# Autodesk Inventor assembly: Ensamblaje1
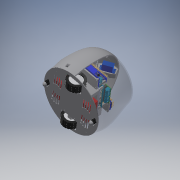
[picture p0: Inventor's stored thumbnail of the model, 180x180]
Saved by Autodesk Inventor 2018 (Build 220112000, 112)
## iProperties
Created: 2018-02-22
Part Number: Ensamblaje1
Material: Genérico
Document SubType Name: Assembly
Designer: ivanb
Author: ivanb
## Documents named in this file (22)
- C:\Users\ivanb\learnbot-git-annex\learnbot_desings\Learnbot2.1\IPT\Learnbot2.0.iam
- C:\Users\ivanb\learnbot-git-annex\learnbot_desings\Learnbot2.1\IPT\Base.ipt
- C:\Users\ivanb\learnbot-git-annex\learnbot_desings\Learnbot2.1\IPT\BackCase.ipt
- C:\Users\ivanb\learnbot-git-annex\learnbot_desings\Learnbot2.1\IPT\Front Case.ipt
- C:\Users\ivanb\learnbot-git-annex\learnbot_desings\Learnbot2.0\filesToPrintLearnbot\IPT\carcasa_camara2.0.ipt
- C:\Users\ivanb\learnbot-git-annex\servo motor.ipt
- C:\Users\ivanb\learnbot-git-annex\learnbot_desings\Learnbot2.1\IPT\Wheel.ipt
- C:\Users\ivanb\learnbot-git-annex\learnbot_desings\Learnbot2.1\IPT\Caster ball.ipt
- C:\Users\ivanb\learnbot-git-annex\learnbot_desings\Learnbot2.1\IPT\Servo Pulley.ipt
- C:\Users\ivanb\learnbot-git-annex\learnbot_desings\Learnbot2.1\IPT\Cover camera case.ipt
- C:\Users\ivanb\learnbot-git-annex\learnbot_desings\Learnbot2.1\IPT\raspberrypi.ipt
- C:\Users\ivanb\learnbot-git-annex\learnbot_desings\Learnbot2.1\IPT\Soport Raspberry.ipt
- C:\Users\ivanb\learnbot-git-annex\learnbot_desings\Learnbot2.1\IPT\Pitft 3.5.ipt
- C:\Users\ivanb\learnbot-git-annex\learnbot_desings\Learnbot2.1\IPT\Expansion-Extension.ipt
- C:\Users\ivanb\learnbot-git-annex\learnbot_desings\Learnbot2.1\IPT\Spacer 3mm.ipt
- C:\Users\ivanb\learnbot-git-annex\learnbot_desings\Learnbot2.1\IPT\pololu 8835.ipt
- C:\Users\ivanb\learnbot-git-annex\learnbot_desings\Learnbot2.1\IPT\Voltage regulator.ipt
- C:\Users\ivanb\learnbot-git-annex\learnbot_desings\Learnbot2.1\IPT\Spacer 19.5 mm.ipt
- C:\Users\ivanb\learnbot-git-annex\learnbot_desings\Learnbot2.1\IPT\Pin multiplier.ipt
- C:\Users\ivanb\learnbot-git-annex\learnbot_desings\Learnbot2.1\IPT\Batery.ipt
- C:\Users\ivanb\learnbot-git-annex\learnbot_desings\Learnbot2.1\IPT\Board 16 pwm.ipt
- C:\Users\ivanb\learnbot-git-annex\learnbot_desings\Learnbot2.1\IPT\Soport 16 pwm.ipt
## Components (27 placed, 21 different names)
1. Base:1 — Coincidencia:1, Insertar:1, Insertar:2, Coincidencia:2, Coincidencia:5, Coincidencia:6, Insertar:11, Insertar:12, Insertar:13, Insertar:14, Insertar:29, Insertar:30, Insertar:32, Insertar:33, Insertar:34, Insertar:35, Coincidencia:12
2. Front Case:1 — Coincidencia:1, Insertar:1, Insertar:2, Insertar:6, Insertar:7, Insertar:8, Insertar:10, Insertar:19, Insertar:28, Insertar:29, Insertar:30, Coincidencia:14, Coincidencia:15, Coincidencia:16
3. BackCase:1 — Coincidencia:2, Insertar:32, Insertar:33
4. carcasa_camara2.0:1 — Nivelación:2, Insertar:8, Coincidencia:7, Insertar:9, Insertar:10, Insertar:19, Rígido:3, Insertar:20
5. servo motor:1 — Nivelación:2, Insertar:6, Insertar:7, De rotación:1, Insertar:28
6. Wheel:1 — Rígido:5
7. Wheel:2 — Rígido:4
8. Caster ball:1 — Coincidencia:6, Insertar:11, Insertar:12
9. Caster ball:2 — Coincidencia:5, Insertar:13, Insertar:14
10. Servo Pulley:1 — De rotación:1
11. Cover camera case:1 — Coincidencia:7, Insertar:9, Rígido:3, Insertar:20
12. Pitft 3.5:1 — Coincidencia:14, Coincidencia:15, Coincidencia:16
13. Soport Raspberry:1 — Insertar:34, Insertar:35, Rígido:4, Rígido:5, Insertar:36, Insertar:37, Insertar:50, Insertar:51, Coincidencia:13
14. raspberrypi:1 — Insertar:36, Insertar:37, Tangente:1, Tangente:2, Coincidencia:10, Insertar:38, Insertar:39, Insertar:40, Insertar:41
15. Expansion-Extension:1 — Tangente:1, Tangente:2, Coincidencia:10, Coincidencia:11, Rígido:6, Insertar:52, Insertar:53
16. Spacer 3mm:1 — Insertar:38
17. Spacer 3mm:2 — Insertar:39
18. Spacer 3mm:3 — Insertar:41
19. Spacer 3mm:4 — Insertar:40
20. pololu 8835:1 — Coincidencia:11, Rígido:6
21. Voltage regulator:1 — Insertar:46, Insertar:47, Insertar:50, Insertar:51
22. Spacer 19.5 mm:3 — Insertar:46, Insertar:48
23. Spacer 19.5 mm:4 — Insertar:47, Insertar:49
24. Pin multiplier:1 — Insertar:48, Insertar:49
25. Batery:1 — Coincidencia:12, Coincidencia:13
26. Board 16 pwm:1 — Insertar:54, Insertar:55
27. Soport 16 pwm:1 — Insertar:52, Insertar:53, Insertar:54, Insertar:55
## Relationships (56: Insert 36, Mate 12, WeldJoint 4, Tangent 2, Flush 1, RevoluteJoint 1)
- Coincidencia:1 [Mate]: Base:1 ↔ Front Case:1
- Insertar:1: Base:1 ↔ Front Case:1
- Insertar:2: Base:1 ↔ Front Case:1
- Coincidencia:2 [Mate]: Base:1 ↔ BackCase:1
- Nivelación:2 [Flush]: carcasa_camara2.0:1 ↔ servo motor:1
- Insertar:6: Front Case:1 ↔ servo motor:1
- Insertar:7: Front Case:1 ↔ servo motor:1
- Coincidencia:5 [Mate]: Base:1 ↔ Caster ball:2
- Coincidencia:6 [Mate]: Base:1 ↔ Caster ball:1
- Insertar:8: Front Case:1 ↔ carcasa_camara2.0:1
- De rotación:1 [RevoluteJoint]: servo motor:1 ↔ Servo Pulley:1
- Coincidencia:7 [Mate]: carcasa_camara2.0:1 ↔ Cover camera case:1
- Insertar:9: carcasa_camara2.0:1 ↔ Cover camera case:1
- Insertar:10: Front Case:1 ↔ carcasa_camara2.0:1
- Insertar:11: Base:1 ↔ Caster ball:1
- Insertar:12: Base:1 ↔ Caster ball:1
- Insertar:13: Base:1 ↔ Caster ball:2
- Insertar:14: Base:1 ↔ Caster ball:2
- Insertar:19: Front Case:1 ↔ carcasa_camara2.0:1
- Rígido:3 [WeldJoint]: carcasa_camara2.0:1 ↔ Cover camera case:1
- Insertar:20: carcasa_camara2.0:1 ↔ Cover camera case:1
- Insertar:28: Front Case:1 ↔ servo motor:1
- Insertar:29: Base:1 ↔ Front Case:1
- Insertar:30: Base:1 ↔ Front Case:1
- Insertar:32: Base:1 ↔ BackCase:1
- Insertar:33: Base:1 ↔ BackCase:1
- Insertar:34: Base:1 ↔ Soport Raspberry:1
- Insertar:35: Base:1 ↔ Soport Raspberry:1
- Rígido:4 [WeldJoint]: Wheel:2 ↔ Soport Raspberry:1
- Rígido:5 [WeldJoint]: Wheel:1 ↔ Soport Raspberry:1
- Insertar:36: Soport Raspberry:1 ↔ raspberrypi:1
- Insertar:37: Soport Raspberry:1 ↔ raspberrypi:1
- Tangente:1: raspberrypi:1 ↔ Expansion-Extension:1
- Tangente:2: raspberrypi:1 ↔ Expansion-Extension:1
- Coincidencia:10 [Mate]: raspberrypi:1 ↔ Expansion-Extension:1
- Insertar:38: raspberrypi:1 ↔ Spacer 3mm:1
- Insertar:39: raspberrypi:1 ↔ Spacer 3mm:2
- Insertar:40: raspberrypi:1 ↔ Spacer 3mm:4
- Insertar:41: raspberrypi:1 ↔ Spacer 3mm:3
- Coincidencia:11 [Mate]: Expansion-Extension:1 ↔ pololu 8835:1
- Rígido:6 [WeldJoint]: Expansion-Extension:1 ↔ pololu 8835:1
- Insertar:46: Voltage regulator:1 ↔ Spacer 19.5 mm:3
- Insertar:47: Voltage regulator:1 ↔ Spacer 19.5 mm:4
- Insertar:48: Spacer 19.5 mm:3 ↔ Pin multiplier:1
- Insertar:49: Spacer 19.5 mm:4 ↔ Pin multiplier:1
- Insertar:50: Soport Raspberry:1 ↔ Voltage regulator:1
- Insertar:51: Soport Raspberry:1 ↔ Voltage regulator:1
- Coincidencia:12 [Mate]: Base:1 ↔ Batery:1
- Coincidencia:13 [Mate]: Soport Raspberry:1 ↔ Batery:1
- Coincidencia:14 [Mate]: Front Case:1 ↔ Pitft 3.5:1
- Coincidencia:15 [Mate]: Front Case:1 ↔ Pitft 3.5:1
- Coincidencia:16 [Mate]: Front Case:1 ↔ Pitft 3.5:1
- Insertar:52: Expansion-Extension:1 ↔ Soport 16 pwm:1
- Insertar:53: Expansion-Extension:1 ↔ Soport 16 pwm:1
- Insertar:54: Board 16 pwm:1 ↔ Soport 16 pwm:1
- Insertar:55: Board 16 pwm:1 ↔ Soport 16 pwm:1
